# Autodesk Inventor assembly: TFVEM_120M
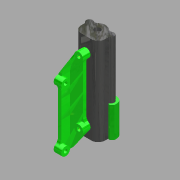
[picture p0: Inventor's stored thumbnail of the model, 180x180]
Saved by Autodesk Inventor 2021 (Build 250183000, 183)
## iProperties
Created: 2021-11-14
Part Number: TFVEM_120M
Document SubType Name: Assembly
Designer: Oliver Ungerer
KODE_ZEICHNUNGSNUMMER: TFVEM_120M
BENENNUNG: Kraftlimitierung
BEARBEITER_NAME: Ungerer O.
MATERIAL: PLA gruen
MASSE: 0.070963
PDMREV: 0+
PROI_VERSION: 0+
PTC_MODIFIED: True
PROI_CREATED_BY: Kantioler_adm
PROI_CREATED_ON: 07.03.2008 12:11:19
PROI_LOCATION: Root-Ordner/Pro_stds/Start_Files
EINHEIT: ST
HERSTELLER_PREIS: 0.0
PRUEFER_NAME: Uo
PTC_ORGANIZATION_ID: Durst
PTC_WM_ITERATION: 0
PTC_WM_VERSION: .0
PTC_WM_CREATED_ON: 10.10.21
PTC_WM_MODIFIED_ON: 10.10.21
AEND_INDEX: 0
PROI_MODIFIED: 1
Author: Oliver Ungerer
## Documents named in this file (5)
- E:\Dokumente\MCI-Mechatronik\Master\Semester_3\Projekt2_CAD\102_Vereinzelung\202.001.02_Kraftlimitierung.iam
- E:\Dokumente\MCI-Mechatronik\Master\Semester_3\Projekt2_CAD\102_Vereinzelung\TFVEM_1200.ipt
- E:\Dokumente\MCI-Mechatronik\Master\Semester_3\Projekt2_CAD\102_Vereinzelung\TFVEM_1201.ipt
- E:\Dokumente\MCI-Mechatronik\Master\Semester_3\Projekt2_CAD\102_Vereinzelung\TFVEM_1202.ipt
- E:\Dokumente\MCI-Mechatronik\Master\Semester_3\Projekt2_CAD\102_Vereinzelung\TFVEM_1203.ipt
## Components (4 placed, 4 different names)
1. TFVEM_1200 — Passend:1, Passend:2, Passend:3, Passend:4, Passend:5, Passend:6, Passend:7, Fluchtend:1
2. TFVEM_1201 — Passend:6, Passend:7, Fluchtend:1
3. TFVEM_1202 — Passend:1, Passend:2, Passend:3
4. TFVEM_1203 — Passend:4, Passend:5
## Relationships (8: Mate 7, Flush 1)
- Passend:1 [Mate]: TFVEM_1200 ↔ TFVEM_1202
- Passend:2 [Mate]: TFVEM_1200 ↔ TFVEM_1202
- Passend:3 [Mate]: TFVEM_1200 ↔ TFVEM_1202
- Passend:4 [Mate]: TFVEM_1200 ↔ TFVEM_1203
- Passend:5 [Mate]: TFVEM_1200 ↔ TFVEM_1203
- Passend:6 [Mate]: TFVEM_1200 ↔ TFVEM_1201
- Passend:7 [Mate]: TFVEM_1200 ↔ TFVEM_1201
- Fluchtend:1 [Flush]: TFVEM_1200 ↔ TFVEM_1201
